# Autodesk Inventor assembly: tower1
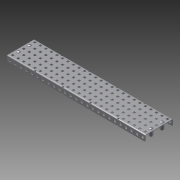
[picture p0: Inventor's stored thumbnail of the model, 180x180]
Saved by Autodesk Inventor 2014 (Build 180170000, 170)
## iProperties
Created: 2013-08-29
Part Number: tower1
Document SubType Name: Assembly
Designer: Ryan
Author: Ryan
## Documents named in this file (4)
- C:\Users\Ryan\Desktop\sw\toss up tower\back support.iam
- C:\Users\Ryan\Desktop\sw\lib\Aperture VEX CAD Library\Hardware\8-32\8-32_.375.ipt
- C:\Users\Ryan\Desktop\sw\lib\Aperture VEX CAD Library\Standoffs\BEAM-0500.ipt
- C:\Users\Ryan\Desktop\sw\lib\Aperture VEX CAD Library\Metal\C Channel\5 x 25.ipt
## Components (9 placed, 3 different names)
1. 5 x 25:1 — Mate:65, Mate:66, Mate:67, Mate:68
2. 8-32_.375:4 — Mate:63, Mate:65, Mate:66, Mate:67
3. BEAM-0500:3 — Mate:63, Mate:68
4. 8-32_.375:5
5. BEAM-0500:4
6. 8-32_.375:6
7. BEAM-0500:5
8. 8-32_.375:7
9. BEAM-0500:6
## Component patterns: (2 elements), (2 elements, first: 8-32_.375:4 + BEAM-0500:3), Component Pattern 10:2 (2 elements)
## Relationships (5: Mate 5)
- Mate:63: 8-32_.375:4 ↔ BEAM-0500:3
- Mate:65: 5 x 25:1 ↔ 8-32_.375:4
- Mate:66 (2.3114 mm): 5 x 25:1 ↔ 8-32_.375:4
- Mate:67 (2.3114 mm): 5 x 25:1 ↔ 8-32_.375:4
- Mate:68: 5 x 25:1 ↔ BEAM-0500:3
## Named parameters: q = 2.3114 mm
